# Autodesk Inventor assembly: 2M1Medytowane złożenie
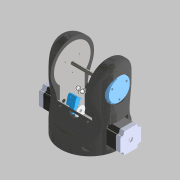
[picture p0: Inventor's stored thumbnail of the model, 180x180]
Saved by Autodesk Inventor 2021 (Build 250183000, 183)
## iProperties
Created: 2021-09-03
Part Number: 2M1Medytowane złożenie
Document SubType Name: Assembly
Designer: marci
Mass: 3863.43 g
Surface Area: 3817.25 cm^2
Volume: 1552.03 cm^3
Density: 2.48928 g/cm^3
Author: marci
## Documents named in this file (23)
- C:\Users\marci\Desktop\Projekt ramienia\2M1\RR-PCSS-2021-2M1.iam
- C:\Users\marci\Desktop\Projekt ramienia\2M1\RR-PCSS-2021-2M1Da.ipt
- C:\Users\marci\Desktop\Projekt ramienia\BCN3D-Moveo-master\CAD files\Nema 23.ipt
- C:\Users\marci\Desktop\Projekt ramienia\BCN3D-Moveo-master\CAD files\Tensor I.iam
- C:\Users\marci\Desktop\Projekt ramienia\Nowy folder\pl-PL\DIN 9021\DIN 9021 - 3,2.ipt
- C:\Users\marci\Desktop\Projekt ramienia\BCN3D-Moveo-master\CAD files\Tensor D.iam
- C:\Users\marci\Desktop\Projekt ramienia\Nowy folder\pl-PL\ISO 7380-1\ISO 7380-1 - M3 x 30.ipt
- C:\Users\marci\Desktop\Projekt ramienia\Nowy folder\pl-PL\ISO 4035(2)\ISO 4035 - M3 - ISO.ipt
- C:\Users\marci\Desktop\Projekt ramienia\Nowy folder\pl-PL\DIN 9021\DIN 9021 - 5,3.ipt
- C:\Users\marci\Desktop\Projekt ramienia\Nowy folder\pl-PL\ISO 4762(2)\ISO 4762 - M5 x 20ISO.ipt
- C:\Users\marci\Desktop\Projekt ramienia\Nowy folder\pl-PL\ISO 4036(2)\ISO 4036 - M5(2).ipt
- C:\Users\marci\Desktop\Projekt ramienia\Nowy folder\pl-PL\ISO 7046-1 H(1)\ISO 7046-1 - M5 x 20 - 4.8 - H - ISO.ipt
- C:\Users\marci\Desktop\Projekt ramienia\Nowy folder\pl-PL\DIN EN 24 036(2)\DIN EN 24 036 - M5.ipt
- C:\Users\marci\Desktop\Projekt ramienia\BCN3D-Moveo-master\CAD files\8mm Bearing.ipt
- C:\Users\marci\Desktop\Projekt ramienia\BCN3D-Moveo-master\CAD files\Tapa 2M1C.ipt
- C:\Users\marci\Desktop\Projekt ramienia\Nowy folder\pl-PL\ISO 4762(2)\ISO 4762 - M3 x 25ISO.ipt
- C:\Users\marci\Desktop\Projekt ramienia\2M1\RR-PCSS-2021-2M1Db.ipt
- C:\Users\marci\Desktop\Projekt ramienia\Nowy folder\pl-PL\ISO 4762(2)\ISO 4762 - M8 x 70ISO.ipt
- C:\Users\marci\Desktop\Projekt ramienia\Nowy folder\pl-PL\ISO 4035(2)\ISO 4035 - M8 - ISO.ipt
- C:\Users\marci\Desktop\Projekt ramienia\2M1\RR-PCSS-2021-W2M1.iam
- C:\Users\marci\Desktop\Projekt ramienia\2M1\Pulley 8mm IGNIS.ipt
- C:\Users\marci\Desktop\Projekt ramienia\Nowy folder\pl-PL\ISO 4161\ISO 4161 - M8(1).ipt
- C:\Users\marci\Desktop\Projekt ramienia\Nowy folder\pl-PL\ANSI B18.3.1M(6)\ANSI B18.3.1M - M8x1,25 x 140(1).ipt
## Components (53 placed, 22 different names)
1. RR-PCSS-2021-2M1Da:1 — Wstawiające:1, Zestawiające:7, Zestawiające:28, Zestawiające:29, Zestawiające:30, Zestawiające:31, Zestawiające:32, Równoległe:2, Zestawiające:61, Zestawiające:63, Wstawiające:18, Równoległe:3, Zestawiające:69
2. Nema 23:1 — Wstawiające:1, Zestawiające:10, Zestawiające:11, Zestawiające:12, Zestawiające:13, Zestawiające:14, Zestawiające:15, Zestawiające:18, Zestawiające:20, Zestawiające:22, Zestawiające:25, Wstawiające:19
3. Nema 23:2 — Wstawiające:16, Wstawiające:20
4. Tensor I:2 [sub-assembly] — Wstawiające:6, Zestawiające:5
5. DIN 9021 3,2:1 — Wstawiające:7
6. DIN 9021 3,2:2 — Wstawiające:6
7. Tensor D:1 [sub-assembly] — Wstawiające:7, Zestawiające:5, Zestawiające:9
8. ISO 7380-1 M3 x 30:1 — Zestawiające:7
9. ISO 4035 M3:1 — Zestawiające:9
10. ISO 4762 M5 x 20:1 — Zestawiające:10, Zestawiające:11
11. DIN 9021 5,3:1 — Zestawiające:18, Wstawiające:8
12. ISO 4036 M5:1 — Wstawiające:8
13. ISO 4762 M5 x 20:2 — Zestawiające:12, Zestawiające:13
14. ISO 4762 M5 x 20:3 — Zestawiające:14, Zestawiające:15
15. DIN 9021 5,3:2 — Zestawiające:20, Wstawiające:9
16. DIN 9021 5,3:3 — Zestawiające:22, Wstawiające:10
17. ISO 4036 M5:2 — Wstawiające:9
18. ISO 4036 M5:3 — Wstawiające:10
19. ISO 7046-1 H M5 x 20 - 4.8 - H:1
20. DIN EN 24036 M5:1 — Zestawiające:25
21. ISO 7380-1 M3 x 30:2
22. ISO 4035 M3:2
23. ISO 4762 M5 x 20:4
24. DIN 9021 5,3:4
25. ISO 4036 M5:4
26. ISO 4762 M5 x 20:5
27. ISO 4762 M5 x 20:6
28. DIN 9021 5,3:5
29. DIN 9021 5,3:6
30. ISO 4036 M5:5
31. ISO 4036 M5:6
32. ISO 7046-1 H M5 x 20 - 4.8 - H:2
33. DIN EN 24036 M5:2
34. 8mm Bearing:1 — Zestawiające:28, Zestawiające:29, Zestawiające:70, Zestawiające:71, Zestawiające:72
35. 8mm Bearing:2 — Wstawiające:17, Zestawiające:73
36. Tapa 2M1C:1 — Zestawiające:48, Zestawiające:49, Zestawiające:50, Zestawiające:51, Zestawiające:52, Zestawiające:53, Zestawiające:59
37. Tapa 2M1C:2 — Zestawiające:30, Zestawiające:31, Zestawiające:32, Zestawiające:42, Zestawiające:43, Zestawiające:44, Zestawiające:45, Zestawiające:46, Zestawiające:47
38. ISO 4762 M3 x 25:4 — Zestawiające:48, Zestawiające:49, Zestawiające:57
39. ISO 4762 M3 x 25:1 — Zestawiające:42, Zestawiające:43
40. ISO 4762 M3 x 25:2 — Zestawiające:44, Zestawiające:45
41. ISO 4762 M3 x 25:3 — Zestawiające:46, Zestawiające:47
42. ISO 4762 M3 x 25:5 — Zestawiające:50, Zestawiające:51
43. ISO 4762 M3 x 25:6 — Zestawiające:52, Zestawiające:53, Zestawiające:58
44. RR-PCSS-2021-2M1Db:1 — Równoległe:2, Wstawiające:16, Wstawiające:17, Zestawiające:57, Zestawiające:58, Zestawiające:59, Zestawiające:60, Zestawiające:62, Zestawiające:64, Zestawiające:65, Zestawiające:66, Zestawiające:67, Zestawiające:68, Równoległe:4, Zestawiające:69
45. ISO 4762 M8 x 70:1 — Zestawiające:60, Zestawiające:61
46. ISO 4035 M8:1 — Zestawiające:64, Zestawiające:65
47. ISO 4762 M8 x 70:2 — Zestawiające:62, Zestawiające:63
48. ISO 4035 M8:2 — Zestawiające:66, Zestawiające:67
49. RR-PCSS-2021-W2M1:1 [sub-assembly] — Zestawiające:68, Wstawiające:18, Równoległe:3, Równoległe:4
50. Pulley 8mm IGNIS:1 — Wstawiające:19
51. Pulley 8mm IGNIS:2 — Wstawiające:20
52. Wkręt z łbem o zmniejszonych wymiarach z gniazdem kutym - Metryczny M8x1,25 x 140:1 — Zestawiające:70, Zestawiające:71
53. ISO 4161 M8:1 — Zestawiające:72, Zestawiające:73
## Relationships (61: Mate 47, Insert 11, Flush 3)
- Wstawiające:1 [Insert]: RR-PCSS-2021-2M1Da:1 ↔ Nema 23:1
- Wstawiające:6 [Insert]: Tensor I:2 ↔ DIN 9021 3,2:2
- Wstawiające:7 [Insert]: DIN 9021 3,2:1 ↔ Tensor D:1
- Zestawiające:5 [Mate]: Tensor I:2 ↔ Tensor D:1
- Zestawiające:7 [Mate]: RR-PCSS-2021-2M1Da:1 ↔ ISO 7380-1 M3 x 30:1
- Zestawiające:9 [Mate]: Tensor D:1 ↔ ISO 4035 M3:1
- Zestawiające:10 [Mate]: Nema 23:1 ↔ ISO 4762 M5 x 20:1
- Zestawiające:11 [Mate]: Nema 23:1 ↔ ISO 4762 M5 x 20:1
- Zestawiające:12 [Mate]: Nema 23:1 ↔ ISO 4762 M5 x 20:2
- Zestawiające:13 [Mate]: Nema 23:1 ↔ ISO 4762 M5 x 20:2
- Zestawiające:14 [Mate]: Nema 23:1 ↔ ISO 4762 M5 x 20:3
- Zestawiające:15 [Mate]: Nema 23:1 ↔ ISO 4762 M5 x 20:3
- Zestawiające:18 [Mate]: Nema 23:1 ↔ DIN 9021 5,3:1
- Zestawiające:20 [Mate]: Nema 23:1 ↔ DIN 9021 5,3:2
- Zestawiające:22 [Mate]: Nema 23:1 ↔ DIN 9021 5,3:3
- Wstawiające:8 [Insert]: DIN 9021 5,3:1 ↔ ISO 4036 M5:1
- Wstawiające:9 [Insert]: DIN 9021 5,3:2 ↔ ISO 4036 M5:2
- Wstawiające:10 [Insert]: DIN 9021 5,3:3 ↔ ISO 4036 M5:3
- Zestawiające:25 [Mate]: Nema 23:1 ↔ DIN EN 24036 M5:1
- Zestawiające:28 [Mate]: RR-PCSS-2021-2M1Da:1 ↔ 8mm Bearing:1
- Zestawiające:29 [Mate]: RR-PCSS-2021-2M1Da:1 ↔ 8mm Bearing:1
- Zestawiające:30 [Mate]: RR-PCSS-2021-2M1Da:1 ↔ Tapa 2M1C:2
- Zestawiające:31 [Mate]: RR-PCSS-2021-2M1Da:1 ↔ Tapa 2M1C:2
- Zestawiające:32 [Mate]: RR-PCSS-2021-2M1Da:1 ↔ Tapa 2M1C:2
- Zestawiające:42 [Mate]: Tapa 2M1C:2 ↔ ISO 4762 M3 x 25:1
- Zestawiające:43 [Mate]: Tapa 2M1C:2 ↔ ISO 4762 M3 x 25:1
- Zestawiające:44 [Mate]: Tapa 2M1C:2 ↔ ISO 4762 M3 x 25:2
- Zestawiające:45 [Mate]: Tapa 2M1C:2 ↔ ISO 4762 M3 x 25:2
- Zestawiające:46 [Mate]: Tapa 2M1C:2 ↔ ISO 4762 M3 x 25:3
- Zestawiające:47 [Mate]: Tapa 2M1C:2 ↔ ISO 4762 M3 x 25:3
- Zestawiające:48 [Mate]: Tapa 2M1C:1 ↔ ISO 4762 M3 x 25:4
- Zestawiające:49 [Mate]: Tapa 2M1C:1 ↔ ISO 4762 M3 x 25:4
- Zestawiające:50 [Mate]: Tapa 2M1C:1 ↔ ISO 4762 M3 x 25:5
- Zestawiające:51 [Mate]: Tapa 2M1C:1 ↔ ISO 4762 M3 x 25:5
- Zestawiające:52 [Mate]: Tapa 2M1C:1 ↔ ISO 4762 M3 x 25:6
- Zestawiające:53 [Mate]: Tapa 2M1C:1 ↔ ISO 4762 M3 x 25:6
- Równoległe:2 [Flush]: RR-PCSS-2021-2M1Da:1 ↔ RR-PCSS-2021-2M1Db:1
- Wstawiające:16 [Insert]: Nema 23:2 ↔ RR-PCSS-2021-2M1Db:1
- Wstawiające:17 [Insert]: 8mm Bearing:2 ↔ RR-PCSS-2021-2M1Db:1
- Zestawiające:57 [Mate]: ISO 4762 M3 x 25:4 ↔ RR-PCSS-2021-2M1Db:1
- Zestawiające:58 [Mate]: ISO 4762 M3 x 25:6 ↔ RR-PCSS-2021-2M1Db:1
- Zestawiające:59 [Mate]: Tapa 2M1C:1 ↔ RR-PCSS-2021-2M1Db:1
- Zestawiające:60 [Mate]: RR-PCSS-2021-2M1Db:1 ↔ ISO 4762 M8 x 70:1
- Zestawiające:61 [Mate]: RR-PCSS-2021-2M1Da:1 ↔ ISO 4762 M8 x 70:1
- Zestawiające:62 [Mate]: RR-PCSS-2021-2M1Db:1 ↔ ISO 4762 M8 x 70:2
- Zestawiające:63 [Mate]: RR-PCSS-2021-2M1Da:1 ↔ ISO 4762 M8 x 70:2
- Zestawiające:64 [Mate]: RR-PCSS-2021-2M1Db:1 ↔ ISO 4035 M8:1
- Zestawiające:65 [Mate]: RR-PCSS-2021-2M1Db:1 ↔ ISO 4035 M8:1
- Zestawiające:66 [Mate]: RR-PCSS-2021-2M1Db:1 ↔ ISO 4035 M8:2
- Zestawiające:67 [Mate]: RR-PCSS-2021-2M1Db:1 ↔ ISO 4035 M8:2
- Zestawiające:68 [Mate]: RR-PCSS-2021-2M1Db:1 ↔ RR-PCSS-2021-W2M1:1
- Wstawiające:18 [Insert]: RR-PCSS-2021-2M1Da:1 ↔ RR-PCSS-2021-W2M1:1
- Równoległe:3 [Flush]: RR-PCSS-2021-2M1Da:1 ↔ RR-PCSS-2021-W2M1:1
- Równoległe:4 [Flush]: RR-PCSS-2021-2M1Db:1 ↔ RR-PCSS-2021-W2M1:1
- Zestawiające:69 [Mate]: RR-PCSS-2021-2M1Da:1 ↔ RR-PCSS-2021-2M1Db:1
- Wstawiające:19 [Insert]: Nema 23:1 ↔ Pulley 8mm IGNIS:1
- Wstawiające:20 [Insert]: Nema 23:2 ↔ Pulley 8mm IGNIS:2
- Zestawiające:70 [Mate]: 8mm Bearing:1 ↔ Wkręt z łbem o zmniejszonych wymiarach z gniazdem kutym - Metryczny M8x1,25 x 140:1
- Zestawiające:71 [Mate]: 8mm Bearing:1 ↔ Wkręt z łbem o zmniejszonych wymiarach z gniazdem kutym - Metryczny M8x1,25 x 140:1
- Zestawiające:72 [Mate]: 8mm Bearing:1 ↔ ISO 4161 M8:1
- Zestawiające:73 [Mate]: 8mm Bearing:2 ↔ ISO 4161 M8:1
